# Autodesk Inventor assembly: MCEN4000:B0
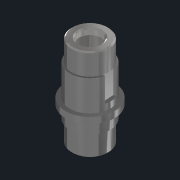
[picture p0: Inventor's stored thumbnail of the model, 180x180]
Saved by Autodesk Inventor 2021 (Build 250183000, 183)
## iProperties
Created: 2020-10-21
Part Number: MCEN4000:B0
Document SubType Name: Assembly
Designer: Eugene Tang
Mass: 2595.01 g
Surface Area: 961.449 cm^2
Volume: 324.843 cm^3
Density: 7.98849 g/cm^3
Description: Ball Nut Assembly
Author: Eugene Tang
## Documents named in this file (5)
- C:\Users\teuge\OneDrive - Curtin University of Technology Australia\Y4S2\DFM\Group Project\CAD\Parts\Assemblies\Ball Screw Ball Assembly.iam
- C:\Users\teuge\OneDrive - Curtin University of Technology Australia\Y4S2\DFM\Group Project\CAD\Master\Ball Screw Nut 1.0.ipt
- C:\Users\teuge\OneDrive - Curtin University of Technology Australia\Y4S2\DFM\Group Project\CAD\Master\BallScrewNut Cap.ipt
- C:\Users\teuge\OneDrive - Curtin University of Technology Australia\Y4S2\DFM\Group Project\CAD\Master\Front Returd Mech.ipt
- C:\Users\teuge\OneDrive - Curtin University of Technology Australia\Y4S2\DFM\Group Project\CAD\Parts\Ball Screw Balls.ipt
## Components (6 placed, 4 different names)
1. Ball Screw Nut 1.0:1 — Mate:1, Mate:2, Mate:3, Mate:4, Mate:5, Mate:6, Mate:7, Mate:8, Mate:9, Mate:10, Mate:11, Mate:12
2. BallScrewNut Cap:1 — Mate:9, Mate:10
3. BallScrewNut Cap:2 — Mate:7, Mate:8
4. Front Returd Mech:1 — Mate:4, Mate:5, Mate:6
5. Front Returd Mech:2 — Mate:1, Mate:2, Mate:3
6. Ball Screw Balls:1 — Mate:11, Mate:12
## Relationships (12: Mate 12)
- Mate:1: Ball Screw Nut 1.0:1 ↔ Front Returd Mech:2
- Mate:2: Ball Screw Nut 1.0:1 ↔ Front Returd Mech:2
- Mate:3: Ball Screw Nut 1.0:1 ↔ Front Returd Mech:2
- Mate:4: Ball Screw Nut 1.0:1 ↔ Front Returd Mech:1
- Mate:5: Ball Screw Nut 1.0:1 ↔ Front Returd Mech:1
- Mate:6: Ball Screw Nut 1.0:1 ↔ Front Returd Mech:1
- Mate:7: Ball Screw Nut 1.0:1 ↔ BallScrewNut Cap:2
- Mate:8: Ball Screw Nut 1.0:1 ↔ BallScrewNut Cap:2
- Mate:9: Ball Screw Nut 1.0:1 ↔ BallScrewNut Cap:1
- Mate:10: Ball Screw Nut 1.0:1 ↔ BallScrewNut Cap:1
- Mate:11: Ball Screw Nut 1.0:1 ↔ Ball Screw Balls:1
- Mate:12: Ball Screw Nut 1.0:1 ↔ Ball Screw Balls:1
## Named parameters: d3_1 = 82.872505 deg
